# Autodesk Inventor assembly: zlozenie_nowe
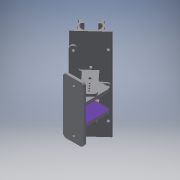
[picture p0: Inventor's stored thumbnail of the model, 180x180]
Saved by Autodesk Inventor 2017 (Build 210142000, 142)
## iProperties
Part Number: zlozenie_nowe
Material: Ogólny
Document SubType Name: Assembly
Designer: patry
Author: patry
## Documents named in this file (4)
- C:\Users\patry\Desktop\realsens\mocowanie\zlozenie_nowe.iam
- C:\Users\patry\Desktop\realsens\mocowanie\czesc_do_obudowy.ipt
- C:\Users\patry\Desktop\realsens\mocowanie\Czesc_do_Ramy.ipt
- C:\Users\patry\Desktop\realsens\mocowanie\test_obudowa.ipt
## Components (3 placed, 3 different names)
1. czesc_do_obudowy:1 — Wstaw:1, Wstaw:2, Wstaw:3
2. Czesc_do_Ramy:1 — Wstaw:3
3. test_obudowa:1 — Wstaw:1, Wstaw:2
## Relationships (3: Insert 3)
- Wstaw:1 [Insert]: czesc_do_obudowy:1 ↔ test_obudowa:1
- Wstaw:2 [Insert]: czesc_do_obudowy:1 ↔ test_obudowa:1
- Wstaw:3 [Insert]: czesc_do_obudowy:1 ↔ Czesc_do_Ramy:1
